# Autodesk Inventor assembly: Ensamblaje_engranes
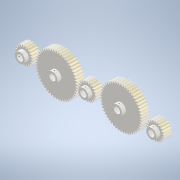
[picture p0: Inventor's stored thumbnail of the model, 180x180]
Saved by Autodesk Inventor 2021 (Build 250183000, 183)
## iProperties
Created: 2021-02-06
Part Number: Ensamblaje_engranes
Document SubType Name: Assembly
Designer: rotje
Author: rotje
## Documents named in this file (3)
- C:\Users\rotje\Documents\Inventor\MSF\Ensamblaje_engranes.iam
- C:\Users\rotje\Documents\Inventor\MSF\Engranaje recto_20_Dientes.ipt
- C:\Users\rotje\Documents\Inventor\MSF\Engranaje recto_50_Dientes.ipt
## Components (5 placed, 2 different names)
1. Engranaje recto1:1 — Coincidencia:1, Coincidencia:2
2. Engranaje recto2:1 — Coincidencia:3
3. Engranaje recto1:3 — Coincidencia:4
4. Engranaje recto1:2 — Coincidencia:6
5. Engranaje recto2:2 — Coincidencia:7
## Relationships (6: Mate 6)
- Coincidencia:1 [Mate]: Engranaje recto1:1
- Coincidencia:2 [Mate]: Engranaje recto1:1
- Coincidencia:3 [Mate]: Engranaje recto2:1
- Coincidencia:4 [Mate]: Engranaje recto1:3
- Coincidencia:6 [Mate]: Engranaje recto1:2
- Coincidencia:7 [Mate]: Engranaje recto2:2
